# Autodesk Inventor assembly: MAIN gripper assembly
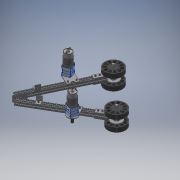
[picture p0: Inventor's stored thumbnail of the model, 180x180]
Saved by Autodesk Inventor 2019 (Build 230136000, 136)
## iProperties
Created: 2019-01-19
Part Number: MAIN gripper assembly
Document SubType Name: Assembly
Designer: Tiberus
Author: Tiberus
## Documents named in this file (7)
- G:\Robotics\Ball Intake 2019\MAIN gripper assembly.iam
- G:\Robotics\Ball Intake 2019\arm assembly left.iam
- G:\Robotics\Ball Intake 2019\arm assembly right.iam
- G:\Robotics\Ball Intake 2019\hinge half.ipt
- C:\Users\Tiberus\Downloads\92196A241_18-8 STAINLESS STEEL SOCKET HEAD CAP SCREW.ipt
- G:\Robotics\Ball Intake 2019\spring extentsion.ipt
- G:\Robotics\Ball Intake 2019\92196A241_18-8 STAINLESS STEEL SOCKET HEAD CAP SCREW.ipt
## Components (16 placed, 5 different names)
1. arm assembly left:1 [sub-assembly] — Mate:2, Flush:2, Flush:3, Mate:7, Mate:8, Mate:9, Mate:10, Mate:19, Mate:20, Mate:21, Mate:22, Mate:25, Flush:7
2. arm assembly right:1 [sub-assembly] — Mate:1, Flush:1, Flush:4, Mate:11, Mate:12, Mate:13, Mate:14, Mate:15, Mate:16, Mate:17, Mate:18, Mate:24, Flush:6
3. hinge half:1 — Mate:2, Flush:2, Flush:3, Mate:3, Mate:4
4. hinge half:2 — Mate:1, Flush:1, Flush:4, Mate:3, Mate:4
5. 92196A241_18-8 STAINLESS STEEL SOCKET HEAD CAP SCREW:1 — Mate:9, Mate:10
6. 92196A241_18-8 STAINLESS STEEL SOCKET HEAD CAP SCREW:2 — Mate:7, Mate:8
7. 92196A241_18-8 STAINLESS STEEL SOCKET HEAD CAP SCREW:3 — Mate:21, Mate:22
8. 92196A241_18-8 STAINLESS STEEL SOCKET HEAD CAP SCREW:4 — Mate:19, Mate:20
9. 92196A241_18-8 STAINLESS STEEL SOCKET HEAD CAP SCREW:5 — Mate:15, Mate:16
10. 92196A241_18-8 STAINLESS STEEL SOCKET HEAD CAP SCREW:6 — Mate:17, Mate:18
11. 92196A241_18-8 STAINLESS STEEL SOCKET HEAD CAP SCREW:7 — Mate:11, Mate:12
12. 92196A241_18-8 STAINLESS STEEL SOCKET HEAD CAP SCREW:8 — Mate:13, Mate:14
13. spring extentsion:1 — Mate:25, Flush:7, Mate:26, Mate:27
14. spring extentsion:2 — Mate:24, Flush:6, Mate:28, Mate:29
15. 92196A241_18-8 STAINLESS STEEL SOCKET HEAD CAP SCREW:9 — Mate:26, Mate:27
16. 92196A241_18-8 STAINLESS STEEL SOCKET HEAD CAP SCREW:10 — Mate:28, Mate:29
## Relationships (32: Mate 26, Flush 6)
- Mate:1: arm assembly right:1 ↔ hinge half:2
- Flush:1: arm assembly right:1 ↔ hinge half:2
- Mate:2: arm assembly left:1 ↔ hinge half:1
- Flush:2: arm assembly left:1 ↔ hinge half:1
- Flush:3: arm assembly left:1 ↔ hinge half:1
- Flush:4: arm assembly right:1 ↔ hinge half:2
- Mate:3: hinge half:1 ↔ hinge half:2
- Mate:4: hinge half:1 ↔ hinge half:2
- Mate:7: arm assembly left:1 ↔ 92196A241_18-8 STAINLESS STEEL SOCKET HEAD CAP SCREW:2
- Mate:8: arm assembly left:1 ↔ 92196A241_18-8 STAINLESS STEEL SOCKET HEAD CAP SCREW:2
- Mate:9: arm assembly left:1 ↔ 92196A241_18-8 STAINLESS STEEL SOCKET HEAD CAP SCREW:1
- Mate:10: arm assembly left:1 ↔ 92196A241_18-8 STAINLESS STEEL SOCKET HEAD CAP SCREW:1
- Mate:11: arm assembly right:1 ↔ 92196A241_18-8 STAINLESS STEEL SOCKET HEAD CAP SCREW:7
- Mate:12: arm assembly right:1 ↔ 92196A241_18-8 STAINLESS STEEL SOCKET HEAD CAP SCREW:7
- Mate:13: arm assembly right:1 ↔ 92196A241_18-8 STAINLESS STEEL SOCKET HEAD CAP SCREW:8
- Mate:14: arm assembly right:1 ↔ 92196A241_18-8 STAINLESS STEEL SOCKET HEAD CAP SCREW:8
- Mate:15: arm assembly right:1 ↔ 92196A241_18-8 STAINLESS STEEL SOCKET HEAD CAP SCREW:5
- Mate:16: arm assembly right:1 ↔ 92196A241_18-8 STAINLESS STEEL SOCKET HEAD CAP SCREW:5
- Mate:17: arm assembly right:1 ↔ 92196A241_18-8 STAINLESS STEEL SOCKET HEAD CAP SCREW:6
- Mate:18: arm assembly right:1 ↔ 92196A241_18-8 STAINLESS STEEL SOCKET HEAD CAP SCREW:6
- Mate:19: arm assembly left:1 ↔ 92196A241_18-8 STAINLESS STEEL SOCKET HEAD CAP SCREW:4
- Mate:20: arm assembly left:1 ↔ 92196A241_18-8 STAINLESS STEEL SOCKET HEAD CAP SCREW:4
- Mate:21: arm assembly left:1 ↔ 92196A241_18-8 STAINLESS STEEL SOCKET HEAD CAP SCREW:3
- Mate:22: arm assembly left:1 ↔ 92196A241_18-8 STAINLESS STEEL SOCKET HEAD CAP SCREW:3
- Mate:24: arm assembly right:1 ↔ spring extentsion:2
- Flush:6: arm assembly right:1 ↔ spring extentsion:2
- Mate:25: arm assembly left:1 ↔ spring extentsion:1
- Flush:7: arm assembly left:1 ↔ spring extentsion:1
- Mate:26: spring extentsion:1 ↔ 92196A241_18-8 STAINLESS STEEL SOCKET HEAD CAP SCREW:9
- Mate:27: spring extentsion:1 ↔ 92196A241_18-8 STAINLESS STEEL SOCKET HEAD CAP SCREW:9
- Mate:28: spring extentsion:2 ↔ 92196A241_18-8 STAINLESS STEEL SOCKET HEAD CAP SCREW:10
- Mate:29: spring extentsion:2 ↔ 92196A241_18-8 STAINLESS STEEL SOCKET HEAD CAP SCREW:10
